# Autodesk Inventor assembly: ATX-12V-6-Pin
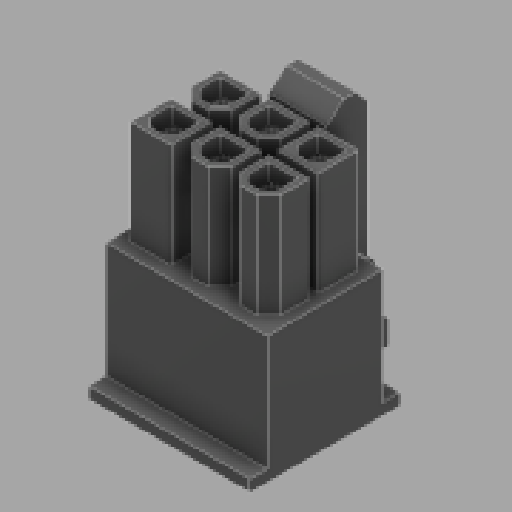
[picture p0: Inventor's stored thumbnail of the model, 512x512]
Saved by Autodesk Inventor 2025 (Build 290162000, 162)
## iProperties
Created: 2015-07-22
Part Number: ATX-12V-6-Pin
Description: STEP AP214
Document SubType Name: Assembly
Designer: Artem Sannikov
Title: ATX-12V-6-Pin.STEP
Revision Number: ANY
Sending System: SolidWorks 2015
Preprocessor: SwSTEP 2.0
## Documents named in this file (4)
- C:\Users\Artem Sannikov\Desktop\Two_axis_gimbal\3D_модели\Основная сборка\ATX-12V-6-Pin.iam
- C:\Users\Artem Sannikov\Desktop\Two_axis_gimbal\3D_модели\Основная сборка\ATX-12V-6-Pin-Body.ipt
- C:\Users\Artem Sannikov\Desktop\Two_axis_gimbal\3D_модели\Основная сборка\ATX-Main-24-Pin-crimp.ipt
- C:\Users\Artem Sannikov\Desktop\Two_axis_gimbal\3D_модели\Провода мотора.ipt
## Components (8 placed, 8 different names)
1. ATX-12V-6-Pin-Body_1
2. ATX-Main-24-Pin-crimp_2
3. ATX-Main-24-Pin-crimp_3 — Заподлицо:1
4. ATX-Main-24-Pin-crimp_4
5. ATX-Main-24-Pin-crimp_5
6. ATX-Main-24-Pin-crimp_6
7. ATX-Main-24-Pin-crimp_7
8. Провода мотора:1 — Заподлицо:1
## Relationships (1: Flush 1)
- Заподлицо:1 [Flush]: ATX-Main-24-Pin-crimp_3 ↔ Провода мотора:1
